# Autodesk Inventor assembly: BallGuideAsmy
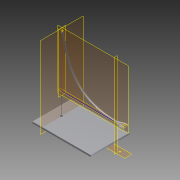
[picture p0: Inventor's stored thumbnail of the model, 180x180]
Saved by Autodesk Inventor 2012 SP2 (Build 160219200, 219)
## iProperties
Created: 2013-07-29
Part Number: BallGuideAsmy
Document SubType Name: Assembly
Designer: 1
Author: 1
## Documents named in this file (3)
- D:\p3_metod1580library\figures\sources\M4-BallDevice\BallGuideAsmy.iam
- D:\p3_metod1580library\figures\sources\M4-BallDevice\BallGuide.ipt
- D:\p3_metod1580library\figures\sources\M4-BallDevice\GuideStand.ipt
## Components (2 placed, 2 different names)
1. BallGuide:1
2. GuideStand:1
## Relationships (1: Flush 1)
- [Flush]: GuideStand:1
